# Autodesk Inventor assembly: FastBattery
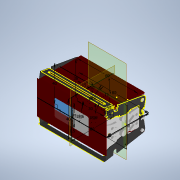
[picture p0: Inventor's stored thumbnail of the model, 180x180]
Saved by Autodesk Inventor 2022 (Build 260153000, 153)
## iProperties
Created: 2024-07-22
Part Number: FastBattery
Document SubType Name: Assembly
Designer: Капустяник Андрей
Author: Капустяник Андрей
## Documents named in this file (16)
- C:\Users\akap\Documents\Git\MZCAT_battery\FastBattery.iam
- C:\Users\akap\Documents\Git\MZCAT_battery\plan.ipt
- C:\Users\akap\Documents\Git\MZCAT_battery\Bat18650.ipt
- C:\Users\akap\Documents\Git\MZCAT_battery\battery_header 7P.ipt
- C:\Users\akap\Documents\Git\MZCAT_battery\xb-acf005-2r.ipt
- C:\Users\akap\Documents\Git\MZCAT_battery\BMS_board.ipt
- C:\Users\akap\Documents\Git\MZCAT_battery\akkum_base1.ipt
- C:\Users\akap\Documents\Git\MZCAT_battery\metal_body_fixed.ipt
- C:\Users\akap\Documents\Git\MZCAT_battery\metal_cap.ipt
- C:\Users\akap\Documents\Git\MZCAT_battery\ButerBoard.ipt
- C:\Users\akap\Documents\Git\MZCAT_battery\petal.ipt
- C:\Users\akap\Documents\Git\MZCAT_battery\User Library-User Library-DFN5x6_SO8FL-1.ipt
- C:\Users\akap\Documents\Git\MZCAT_battery\akkum_base2.ipt
- C:\Users\akap\Documents\Git\MZCAT_battery\investment nut M2 OD3,2 L2,5.ipt
- C:\Users\akap\Documents\Git\MZCAT_battery\M2 4mm HEX.ipt
- C:\Users\akap\Documents\Git\MZCAT_battery\roll.ipt
## Components (32 placed, 15 different names)
1. plan:1 — Заподлицо:1, Заподлицо:2, Заподлицо:3, Совмещение:4, Совмещение:5, Совмещение:6, Совмещение:9
2. Bat18650:1 — Заподлицо:4, Совмещение:1, Совмещение:2, Совмещение:6
3. Bat18650:2 — Заподлицо:5, Совмещение:3, Совмещение:5
4. Bat18650:3 — Заподлицо:4, Заподлицо:5, Совмещение:3, Совмещение:4
5. battery_header 7P:1 — Совмещение:7, Совмещение:9, Совмещение:12, Совмещение:15
6. xb-acf005-2r:1 — Совмещение:17, Совмещение:18
7. BMS_board:1 — Совмещение:7, Совмещение:10, Совмещение:11, Совмещение:12, Совмещение:15, Заподлицо:14, Совмещение:21, Совмещение:22, С поворотом:7, С поворотом:8, С поворотом:9, С поворотом:10
8. akkum_base1:1 — Заподлицо:7, Заподлицо:8, Заподлицо:9, Совмещение:20, Заподлицо:16, Заподлицо:17, Совмещение:27, С поворотом:1, С поворотом:2, С поворотом:4, Совмещение:30, Совмещение:31, Совмещение:32, Совмещение:33, Совмещение:34, Совмещение:35, Совмещение:36, Совмещение:37, Заподлицо:19
9. metal_body_fixed:1 — Совмещение:36, Совмещение:37, Заподлицо:19
10. metal_cap:1 — Заподлицо:13, С поворотом:11, С поворотом:12
11. ButerBoard:1 — Заподлицо:14, Совмещение:16, Совмещение:17, Совмещение:18, Совмещение:19
12. petal:1 — Совмещение:20, Заподлицо:15, Угол:2, Касательность:1, Касательность:3, Заподлицо:18
13. User Library-User Library-DFN5x6_SO8FL-1:1 — Совмещение:22
14. User Library-User Library-DFN5x6_SO8FL-1:2 — Совмещение:21
15. akkum_base2:1 — Заподлицо:16, Заподлицо:17, Совмещение:25, Совмещение:26, Угол:1, Угол:2, Совмещение:27, С поворотом:3, С поворотом:5, С поворотом:6, Совмещение:28, Совмещение:29
16. petal:2 — Совмещение:25, Совмещение:26, Угол:1, Касательность:2, Касательность:4, Заподлицо:18
17. investment nut M2 OD3,2 L2,5:1 — С поворотом:1
18. investment nut M2 OD3,2 L2,5:2 — С поворотом:6
19. investment nut M2 OD3,2 L2,5:3 — С поворотом:5
20. investment nut M2 OD3,2 L2,5:4 — С поворотом:4
21. investment nut M2 OD3,2 L2,5:5 — С поворотом:3
22. investment nut M2 OD3,2 L2,5:6 — С поворотом:2
23. M2 4mm HEX:1 — С поворотом:7
24. M2 4mm HEX:2 — С поворотом:11
25. M2 4mm HEX:3 — С поворотом:9
26. M2 4mm HEX:4 — С поворотом:12
27. M2 4mm HEX:5 — С поворотом:8
28. M2 4mm HEX:6 — С поворотом:10
29. roll:1 — Совмещение:28, Совмещение:35, Касательность:2
30. roll:2 — Совмещение:29, Совмещение:34, Касательность:1
31. roll:3 — Совмещение:30, Совмещение:32, Касательность:4
32. roll:4 — Совмещение:31, Совмещение:33, Касательность:3
## Relationships (65: Mate 32, Flush 15, RevoluteJoint 12, Tangent 4, Angle 2)
- Заподлицо:1 [Flush]: plan:1
- Заподлицо:2 [Flush]: plan:1
- Заподлицо:3 [Flush]: plan:1
- Заподлицо:4 [Flush]: Bat18650:1 ↔ Bat18650:3
- Заподлицо:5 [Flush]: Bat18650:2 ↔ Bat18650:3
- Совмещение:1 [Mate]: Bat18650:1
- Совмещение:2 [Mate]: Bat18650:1
- Совмещение:3 [Mate]: Bat18650:2 ↔ Bat18650:3
- Совмещение:4 [Mate]: plan:1 ↔ Bat18650:3
- Совмещение:5 [Mate]: plan:1 ↔ Bat18650:2
- Совмещение:6 [Mate]: plan:1 ↔ Bat18650:1
- Совмещение:7 [Mate]: battery_header 7P:1 ↔ BMS_board:1
- Совмещение:9 [Mate]: plan:1 ↔ battery_header 7P:1
- Совмещение:10 [Mate]: BMS_board:1
- Совмещение:11 [Mate]: BMS_board:1
- Совмещение:12 [Mate]: battery_header 7P:1 ↔ BMS_board:1
- Заподлицо:7 [Flush]: akkum_base1:1
- Заподлицо:8 [Flush]: akkum_base1:1
- Заподлицо:9 [Flush]: akkum_base1:1
- Заподлицо:13 [Flush]: metal_cap:1
- Совмещение:15 [Mate]: battery_header 7P:1 ↔ BMS_board:1
- Заподлицо:14 [Flush]: BMS_board:1 ↔ ButerBoard:1
- Совмещение:16 [Mate]: ButerBoard:1
- Совмещение:17 [Mate]: xb-acf005-2r:1 ↔ ButerBoard:1
- Совмещение:18 [Mate]: xb-acf005-2r:1 ↔ ButerBoard:1
- Совмещение:19 [Mate] (-10 mm): ButerBoard:1
- Совмещение:20 [Mate]: akkum_base1:1 ↔ petal:1
- Заподлицо:15 [Flush] (-38.5 mm): petal:1
- Совмещение:21 [Mate]: BMS_board:1 ↔ User Library-User Library-DFN5x6_SO8FL-1:2
- Совмещение:22 [Mate]: BMS_board:1 ↔ User Library-User Library-DFN5x6_SO8FL-1:1
- Заподлицо:16 [Flush]: akkum_base1:1 ↔ akkum_base2:1
- Заподлицо:17 [Flush]: akkum_base1:1 ↔ akkum_base2:1
- Совмещение:25 [Mate]: akkum_base2:1 ↔ petal:2
- Совмещение:26 [Mate] (0.8 mm): akkum_base2:1 ↔ petal:2
- Угол:1 [Angle] (0 deg): akkum_base2:1 ↔ petal:2
- Угол:2 [Angle] (0 deg): petal:1 ↔ akkum_base2:1
- Совмещение:27 [Mate] (0.3 mm): akkum_base1:1 ↔ akkum_base2:1
- С поворотом:1 [RevoluteJoint]: akkum_base1:1 ↔ investment nut M2 OD3,2 L2,5:1
- С поворотом:2 [RevoluteJoint]: akkum_base1:1 ↔ investment nut M2 OD3,2 L2,5:6
- С поворотом:3 [RevoluteJoint]: akkum_base2:1 ↔ investment nut M2 OD3,2 L2,5:5
- С поворотом:4 [RevoluteJoint]: akkum_base1:1 ↔ investment nut M2 OD3,2 L2,5:4
- С поворотом:5 [RevoluteJoint]: akkum_base2:1 ↔ investment nut M2 OD3,2 L2,5:3
- С поворотом:6 [RevoluteJoint]: akkum_base2:1 ↔ investment nut M2 OD3,2 L2,5:2
- С поворотом:7 [RevoluteJoint]: BMS_board:1 ↔ M2 4mm HEX:1
- С поворотом:8 [RevoluteJoint]: BMS_board:1 ↔ M2 4mm HEX:5
- С поворотом:9 [RevoluteJoint]: BMS_board:1 ↔ M2 4mm HEX:3
- С поворотом:10 [RevoluteJoint]: BMS_board:1 ↔ M2 4mm HEX:6
- С поворотом:11 [RevoluteJoint]: metal_cap:1 ↔ M2 4mm HEX:2
- С поворотом:12 [RevoluteJoint]: metal_cap:1 ↔ M2 4mm HEX:4
- Совмещение:28 [Mate]: akkum_base2:1 ↔ roll:1
- Совмещение:29 [Mate]: akkum_base2:1 ↔ roll:2
- Совмещение:30 [Mate]: akkum_base1:1 ↔ roll:3
- Совмещение:31 [Mate]: akkum_base1:1 ↔ roll:4
- Совмещение:32 [Mate]: akkum_base1:1 ↔ roll:3
- Совмещение:33 [Mate]: akkum_base1:1 ↔ roll:4
- Совмещение:34 [Mate]: akkum_base1:1 ↔ roll:2
- Совмещение:35 [Mate]: akkum_base1:1 ↔ roll:1
- Касательность:1 [Tangent]: petal:1 ↔ roll:2
- Касательность:2 [Tangent]: petal:2 ↔ roll:1
- Касательность:3 [Tangent]: petal:1 ↔ roll:4
- Касательность:4 [Tangent]: petal:2 ↔ roll:3
- Заподлицо:18 [Flush]: petal:1 ↔ petal:2
- Совмещение:36 [Mate]: akkum_base1:1 ↔ metal_body_fixed:1
- Совмещение:37 [Mate]: akkum_base1:1 ↔ metal_body_fixed:1
- Заподлицо:19 [Flush]: akkum_base1:1 ↔ metal_body_fixed:1
